# Autodesk Inventor assembly: Right Hook Encoder Assembly
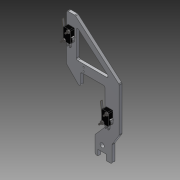
[picture p0: Inventor's stored thumbnail of the model, 180x180]
Saved by Autodesk Inventor 2014 SP1 (Build 180222100, 222)
## iProperties
Created: 2013-03-16
Part Number: Right Hook Encoder Assembly
Document SubType Name: Assembly
Designer: Arpan
Mass: 197.578 g
Surface Area: 360.053 cm^2
Volume: 75.9782 cm^3
Density: 2.60045 g/cm^3
Author: Arpan
## Documents named in this file (6)
- C:\Users\Moses\Documents\Inventor\Sally Rebuild\Rebuild Sally\Right Hook Encoder Assembly.iam
- C:\Users\Moses\Documents\Inventor\Sally Rebuild\Rebuild Sally\7779K630.ipt
- C:\Users\Moses\Documents\Inventor\Sally Rebuild\Rebuild Sally\Rebuild Right Climber Hook.ipt
- C:\Users\Moses\Documents\Inventor\Sally Rebuild\Rebuild Sally\Standard #4 Washer.ipt
- C:\Users\Moses\Documents\Inventor\Sally Rebuild\Rebuild Sally\4-40 18-8 Stainless Steel Pan Head Phillips Machine Screw\1.0000\91772A115.ipt
- C:\Users\Moses\Documents\Inventor\Sally Rebuild\Rebuild Sally\4-40 18-8 Stainless Steel Pan Head Phillips Machine Screw\18-8 Stainless Steel Machine Screw Hex Nut\91841A005.ipt
## Components (17 placed, 5 different names)
1. Rebuild Right Climber Hook:1 — Mate:3, Mate:1, Mate:5, Mate:2, Mate:4, Mate:6, Insert:1, Insert:2, Insert:3, Insert:4, Insert:5, Insert:6
2. 7779K630:1 — Mate:3, Mate:1, Mate:4, Insert:11, Insert:12
3. 7779K630:2 — Mate:5, Mate:2, Mate:6, Insert:13, Insert:14
4. Standard #4 Washer:1 — Insert:1, Insert:7
5. Standard #4 Washer:2 — Insert:2, Insert:8
6. Standard #4 Washer:3 — Insert:3
7. Standard #4 Washer:4 — Insert:4
8. Standard #4 Washer:5 — Insert:5, Insert:9
9. Standard #4 Washer:6 — Insert:6, Insert:10
10. 91772A115:1 — Insert:7
11. 91772A115:2 — Insert:8
12. 91772A115:3 — Insert:9
13. 91772A115:4 — Insert:10
14. 91841A005:1 — Insert:11
15. 91841A005:2 — Insert:12
16. 91841A005:3 — Insert:13
17. 91841A005:4 — Insert:14
## Relationships (20: Insert 14, Mate 6)
- Mate:3: Rebuild Right Climber Hook:1 ↔ 7779K630:1
- Mate:1: Rebuild Right Climber Hook:1 ↔ 7779K630:1
- Mate:5: Rebuild Right Climber Hook:1 ↔ 7779K630:2
- Mate:2: Rebuild Right Climber Hook:1 ↔ 7779K630:2
- Mate:4: Rebuild Right Climber Hook:1 ↔ 7779K630:1
- Mate:6: Rebuild Right Climber Hook:1 ↔ 7779K630:2
- Insert:1: Rebuild Right Climber Hook:1 ↔ Standard #4 Washer:1
- Insert:2: Rebuild Right Climber Hook:1 ↔ Standard #4 Washer:2
- Insert:3: Rebuild Right Climber Hook:1 ↔ Standard #4 Washer:3
- Insert:4: Rebuild Right Climber Hook:1 ↔ Standard #4 Washer:4
- Insert:5: Rebuild Right Climber Hook:1 ↔ Standard #4 Washer:5
- Insert:6: Rebuild Right Climber Hook:1 ↔ Standard #4 Washer:6
- Insert:7: Standard #4 Washer:1 ↔ 91772A115:1
- Insert:8: Standard #4 Washer:2 ↔ 91772A115:2
- Insert:9: Standard #4 Washer:5 ↔ 91772A115:3
- Insert:10: Standard #4 Washer:6 ↔ 91772A115:4
- Insert:11: 7779K630:1 ↔ 91841A005:1
- Insert:12: 7779K630:1 ↔ 91841A005:2
- Insert:13: 7779K630:2 ↔ 91841A005:3
- Insert:14: 7779K630:2 ↔ 91841A005:4
